# Autodesk Inventor assembly: DHT_sestava
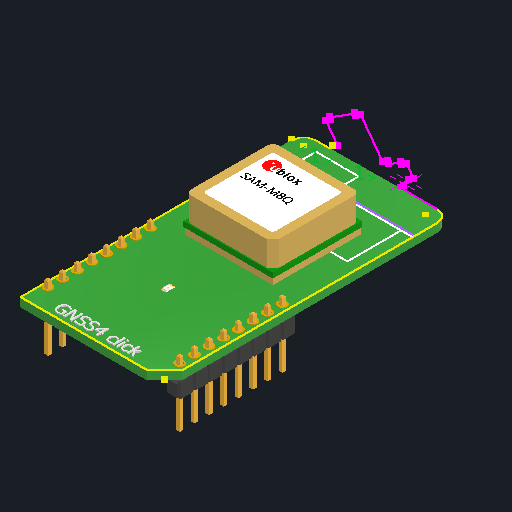
[picture p0: Inventor's stored thumbnail of the model, 512x512]
Saved by Autodesk Inventor 2022 (Build 260153000, 153)
## iProperties
Created: 2022-03-19
Part Number: DHT_sestava
Document SubType Name: Assembly
Designer: dvorakj
Author: dvorakj
## Documents named in this file (5)
- C:\Users\dvorakj\Documents\Inventor\Bakalarka\Clicks\GNSS\GNSS_sestava.iam
- C:\Users\dvorakj\Documents\Inventor\Bakalarka\Clicks\Pin Header\61300811121 (rev1).iam
- C:\Users\dvorakj\Documents\Inventor\Bakalarka\Clicks\GPS\LED\STP_WL-SMCW_150060xx75020 (rev1).iam
- C:\Users\dvorakj\Documents\Inventor\Bakalarka\Clicks\GNSS\GPS_PCB.ipt
- C:\Users\dvorakj\Documents\Inventor\Bakalarka\Clicks\GNSS\Module\GPS_sam-m8q.ipt
## Components (6 placed, 4 different names)
1. 61300811121 (rev1):1 [sub-assembly]
2. 61300811121 (rev1):2 [sub-assembly] — Mate:9, Angle:1, Mate:10
3. STP_WL-SMCW_150060xx75020 (rev1):1 [sub-assembly]
4. STP_WL-SMCW_150060xx75020 (rev1):2 [sub-assembly]
5. GPS_PCB:2 — Mate:9, Angle:1, Mate:10, Mate:11
6. GPS_sam-m8q:1 — Mate:11
## Relationships (4: Mate 3, Angle 1)
- Mate:9: 61300811121 (rev1):2 ↔ GPS_PCB:2
- Angle:1 (0 deg): 61300811121 (rev1):2 ↔ GPS_PCB:2
- Mate:10: 61300811121 (rev1):2 ↔ GPS_PCB:2
- Mate:11: GPS_PCB:2 ↔ GPS_sam-m8q:1
